# Autodesk Inventor assembly: Motherboard_assembly
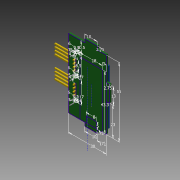
[picture p0: Inventor's stored thumbnail of the model, 180x180]
Saved by Autodesk Inventor 2015 (Build 190159000, 159)
## iProperties
Created: 2015-06-12
Part Number: Motherboard_assembly
Document SubType Name: Assembly
Designer: Openlab
Author: Openlab
## Documents named in this file (4)
- C:\Users\Admin\Alexey\OSS-Spectrophotometer\parts\Motherboard_assembly.iam
- C:\Users\Admin\Alexey\OSS-Spectrophotometer\parts\Motherboard_dummy.ipt
- C:\Users\Admin\Alexey\OSS-Spectrophotometer\parts\Pin-connector-angled-4.iam
- C:\Users\Admin\Alexey\OSS-Spectrophotometer\parts\LED.ipt
## Components (6 placed, 3 different names)
1. Motherboard_dummy:1 — Mate:1, Mate:4, Mate:5, Mate:6, Mate:7, Mate:8, Mate:9, Mate:10, Mate:11, Mate:12, Mate:13, Mate:14
2. Pin-connector-angled-4:1 [sub-assembly] — Mate:1, Mate:7, Mate:8
3. Pin-connector-angled-4:2 [sub-assembly] — Mate:4, Mate:5, Mate:6
4. LED:1 — Mate:9, Mate:10
5. LED:2 — Mate:13, Mate:14
6. LED:3 — Mate:11, Mate:12
## Relationships (12: Mate 12)
- Mate:1: Motherboard_dummy:1 ↔ Pin-connector-angled-4:1
- Mate:4: Motherboard_dummy:1 ↔ Pin-connector-angled-4:2
- Mate:5: Motherboard_dummy:1 ↔ Pin-connector-angled-4:2
- Mate:6: Motherboard_dummy:1 ↔ Pin-connector-angled-4:2
- Mate:7: Motherboard_dummy:1 ↔ Pin-connector-angled-4:1
- Mate:8: Motherboard_dummy:1 ↔ Pin-connector-angled-4:1
- Mate:9: Motherboard_dummy:1 ↔ LED:1
- Mate:10: Motherboard_dummy:1 ↔ LED:1
- Mate:11: Motherboard_dummy:1 ↔ LED:3
- Mate:12: Motherboard_dummy:1 ↔ LED:3
- Mate:13: Motherboard_dummy:1 ↔ LED:2
- Mate:14: Motherboard_dummy:1 ↔ LED:2
